# Autodesk Inventor assembly: Assembly4
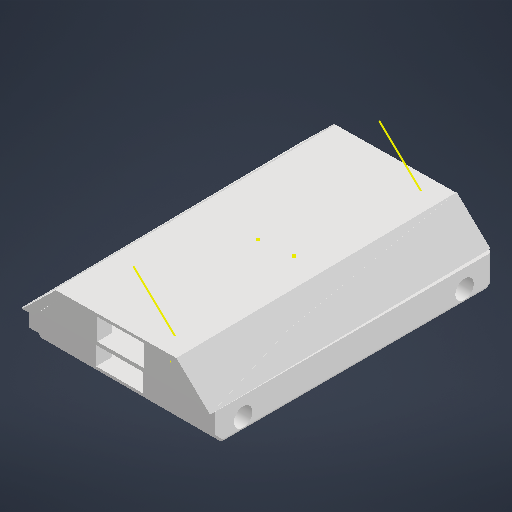
[picture p0: Inventor's stored thumbnail of the model, 512x512]
Saved by Autodesk Inventor 2027 (Build 310192060, 192F)
## iProperties
Created: 2026-06-06
Part Number: Assembly4
Document SubType Name: Assembly
Designer: CatKartikSUPREMEPC
Author: CatKartikSUPREMEPC
## Documents named in this file (3)
- C:\Users\CatKartikSUPREMEPC\Documents\Stasis Design\Assembly4.iam
- C:\Users\CatKartikSUPREMEPC\Documents\Stasis Design\body redesign.ipt
- C:\Users\CatKartikSUPREMEPC\Documents\Stasis Design\cover redesign.ipt
## Components (2 placed, 2 different names)
1. body redesign:1 — Mate:1, Flush:1
2. cover redesign:1 — Mate:1, Flush:1
## Relationships (2: Mate 1, Flush 1)
- Mate:1: body redesign:1 ↔ cover redesign:1
- Flush:1: body redesign:1 ↔ cover redesign:1
